# Autodesk Inventor assembly: Assembly1
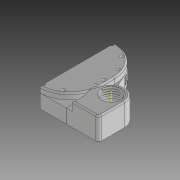
[picture p0: Inventor's stored thumbnail of the model, 180x180]
Saved by Autodesk Inventor 2020 (Build 240168000, 168)
## iProperties
Created: 2021-01-24
Part Number: Assembly1
Document SubType Name: Assembly
Designer: DDeGo
Author: DDeGo
## Documents named in this file (10)
- C:\Users\DDeGo\Documents\Drew\Projects\AirWankelEngine\cad\Assembly1.iam
- C:\Users\DDeGo\Documents\Drew\Projects\AirWankelEngine\cad\housingV2.ipt
- C:\Users\DDeGo\Documents\Drew\Projects\AirWankelEngine\cad\housingValveV2.ipt
- C:\Users\DDeGo\Documents\Drew\Projects\AirWankelEngine\cad\ValveFlapper.ipt
- C:\Users\DDeGo\Documents\Drew\Projects\AirWankelEngine\cad\housingPlate.ipt
- C:\Users\DDeGo\Documents\Drew\Projects\AirWankelEngine\cad\piston.ipt
- C:\Users\DDeGo\Documents\Drew\Projects\AirWankelEngine\cad\6701 bearing.ipt
- C:\Users\DDeGo\Documents\Drew\Projects\AirWankelEngine\cad\MR85 bearing.ipt
- C:\Users\DDeGo\Documents\Drew\Projects\AirWankelEngine\cad\camshaft.ipt
- C:\Users\DDeGo\Documents\Drew\Projects\AirWankelEngine\cad\CamPlate.ipt
## Components (11 placed, 9 different names)
1. housingV2:1 — Flush:1, Mate:1, Flush:2, Mate:2, Mate:3, Mate:4, Mate:5, Mate:6, Mate:9, Mate:10, Mate:14, Mate:15, Mate:18, Mate:19
2. housingValveV2:1 — Flush:1, Mate:1, Flush:2
3. ValveFlapper:1 — Mate:2, Mate:3
4. housingPlate:1 — Mate:4, Mate:5, Mate:6
5. piston:1 — Mate:7, Mate:8, Mate:14
6. 6701 bearing:1 — Mate:7, Mate:8, Mate:13
7. MR85 bearing:1 — Mate:9, Mate:10, Mate:11, Mate:12
8. camshaft:1 — Mate:11, Mate:12, Mate:13, Mate:20, Mate:21
9. CamPlate:1 — Mate:20, Mate:21
10. housingPlate:2 — Mate:15, Mate:16, Mate:17, Mate:18, Mate:19
11. MR85 bearing:2 — Mate:16, Mate:17
## Relationships (23: Mate 21, Flush 2)
- Flush:1: housingV2:1 ↔ housingValveV2:1
- Mate:1: housingV2:1 ↔ housingValveV2:1
- Flush:2: housingV2:1 ↔ housingValveV2:1
- Mate:2: housingV2:1 ↔ ValveFlapper:1
- Mate:3 (0.5 mm): housingV2:1 ↔ ValveFlapper:1
- Mate:4: housingV2:1 ↔ housingPlate:1
- Mate:5: housingV2:1 ↔ housingPlate:1
- Mate:6: housingV2:1 ↔ housingPlate:1
- Mate:7: piston:1 ↔ 6701 bearing:1
- Mate:8: piston:1 ↔ 6701 bearing:1
- Mate:9: housingV2:1 ↔ MR85 bearing:1
- Mate:10: housingV2:1 ↔ MR85 bearing:1
- Mate:11: MR85 bearing:1 ↔ camshaft:1
- Mate:12: MR85 bearing:1 ↔ camshaft:1
- Mate:13: 6701 bearing:1 ↔ camshaft:1
- Mate:14: housingV2:1 ↔ piston:1
- Mate:15: housingV2:1 ↔ housingPlate:2
- Mate:16: housingPlate:2 ↔ MR85 bearing:2
- Mate:17: housingPlate:2 ↔ MR85 bearing:2
- Mate:18: housingV2:1 ↔ housingPlate:2
- Mate:19: housingV2:1 ↔ housingPlate:2
- Mate:20: camshaft:1 ↔ CamPlate:1
- Mate:21: camshaft:1 ↔ CamPlate:1
